# Autodesk Inventor assembly: Assembly1
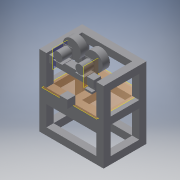
[picture p0: Inventor's stored thumbnail of the model, 180x180]
Saved by Autodesk Inventor 2018 (Build 220112000, 112)
## iProperties
Created: 2019-03-24
Part Number: Assembly1
Document SubType Name: Assembly
Designer: simon
Author: simon
## Documents named in this file (4)
- C:\Users\simon\SynologyDrive\Basteln\2019-05 Badminton Shuttle Feeder\3DModell\Assembly1.iam
- C:\Users\simon\SynologyDrive\Basteln\2019-05 Badminton Shuttle Feeder\3DModell\BSF_Accelerator_v01.ipt
- C:\Users\simon\SynologyDrive\Basteln\2019-05 Badminton Shuttle Feeder\3DModell\BSF_OuterFrame.ipt
- C:\Users\simon\SynologyDrive\Basteln\2019-05 Badminton Shuttle Feeder\3DModell\BSF_ShuttleFeeder.ipt
## Components (3 placed, 3 different names)
1. BSF_Accelerator_v01:1 — Flush:1
2. BSF_OuterFrame:1 — Flush:1, Flush:2, Flush:3, Flush:4
3. BSF_ShuttleFeeder:1 — Flush:2, Flush:3, Flush:4
## Relationships (4: Flush 4)
- Flush:1: BSF_Accelerator_v01:1 ↔ BSF_OuterFrame:1
- Flush:2: BSF_OuterFrame:1 ↔ BSF_ShuttleFeeder:1
- Flush:3: BSF_OuterFrame:1 ↔ BSF_ShuttleFeeder:1
- Flush:4: BSF_OuterFrame:1 ↔ BSF_ShuttleFeeder:1
